# Autodesk Inventor assembly: Samlet Kasse mk2
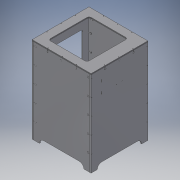
[picture p0: Inventor's stored thumbnail of the model, 180x180]
Saved by Autodesk Inventor 2016 (Build 200138000, 138)
## iProperties
Created: 2015-10-17
Part Number: Samlet Kasse mk2
Document SubType Name: Assembly
Designer: iLyngklip
Author: iLyngklip
## Documents named in this file (7)
- C:\Users\iLyngklip\AppData\Local\Autodesk\Autodesk Sync\Cloud\mathiaslk\UltiBot mk2\Kasse-delene mk2 - Små lejer\Samlet Kasse mk2.iam
- C:\Users\iLyngklip\AppData\Local\Autodesk\Autodesk Sync\Cloud\mathiaslk\UltiBot mk2\Kasse-delene mk2 - Små lejer\Bagsiden mk2.ipt
- C:\Users\iLyngklip\AppData\Local\Autodesk\Autodesk Sync\Cloud\mathiaslk\UltiBot mk2\Kasse-delene mk2 - Små lejer\Forsiden mk2.ipt
- C:\Users\iLyngklip\AppData\Local\Autodesk\Autodesk Sync\Cloud\mathiaslk\UltiBot mk2\Kasse-delene mk2 - Små lejer\Højre side mk2.ipt
- C:\Users\iLyngklip\AppData\Local\Autodesk\Autodesk Sync\Cloud\mathiaslk\UltiBot mk2\Kasse-delene mk2 - Små lejer\Låg mk2.ipt
- C:\Users\iLyngklip\AppData\Local\Autodesk\Autodesk Sync\Cloud\mathiaslk\UltiBot mk2\Kasse-delene mk2 - Små lejer\Mellemplade mk2.ipt
- C:\Users\iLyngklip\AppData\Local\Autodesk\Autodesk Sync\Cloud\mathiaslk\UltiBot mk2\Kasse-delene mk2 - Små lejer\Venstre side mk2.ipt
## Components (6 placed, 6 different names)
1. Bagsiden mk2:1 — Mate:8, Flush:10, Flush:11
2. Forsiden mk2:1 — Flush:2, Flush:1, Mate:2, Flush:3, Mate:3, Flush:4, Flush:6, Flush:9
3. Højre side mk2:1 — Flush:2, Flush:1, Mate:2
4. Låg mk2:1 — Flush:5, Flush:6, Mate:4
5. Mellemplade mk2:1 — Mate:7, Flush:9, Mate:8
6. Venstre side mk2:1 — Flush:3, Mate:3, Flush:4, Flush:5, Mate:4, Mate:7, Flush:10, Flush:11
## Relationships (14: Flush 9, Mate 5)
- Flush:2: Forsiden mk2:1 ↔ Højre side mk2:1
- Flush:1: Forsiden mk2:1 ↔ Højre side mk2:1
- Mate:2: Forsiden mk2:1 ↔ Højre side mk2:1
- Flush:3: Forsiden mk2:1 ↔ Venstre side mk2:1
- Mate:3: Forsiden mk2:1 ↔ Venstre side mk2:1
- Flush:4: Forsiden mk2:1 ↔ Venstre side mk2:1
- Flush:5: Låg mk2:1 ↔ Venstre side mk2:1
- Flush:6: Forsiden mk2:1 ↔ Låg mk2:1
- Mate:4: Låg mk2:1 ↔ Venstre side mk2:1
- Mate:7: Mellemplade mk2:1 ↔ Venstre side mk2:1
- Flush:9 (-54 mm): Forsiden mk2:1 ↔ Mellemplade mk2:1
- Mate:8: Bagsiden mk2:1 ↔ Mellemplade mk2:1
- Flush:10: Bagsiden mk2:1 ↔ Venstre side mk2:1
- Flush:11: Bagsiden mk2:1 ↔ Venstre side mk2:1
